# Autodesk Inventor assembly: CMV12000 Extraction Tool V01
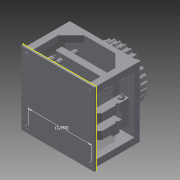
[picture p0: Inventor's stored thumbnail of the model, 180x180]
Saved by Autodesk Inventor 2015 (Build 190159000, 159)
## iProperties
Created: 2016-09-16
Part Number: CMV12000 Extraction Tool V01
Document SubType Name: Assembly
Designer: spichelh
Author: spichelh
## Documents named in this file (7)
- C:\Users\spichelh\Documents\GitHub\beta-hardware\Manufacturing Tools\CMV12000 Extraction Tool V01\CMV12000 Extraction Tool V01.iam
- C:\Users\spichelh\Documents\GitHub\beta-hardware\Manufacturing Tools\CMV12000 Extraction Tool V01\CMV12000v1.ipt
- C:\Users\spichelh\Documents\GitHub\beta-hardware\Manufacturing Tools\CMV12000 Extraction Tool V01\arms01.ipt
- C:\Users\spichelh\Documents\GitHub\beta-hardware\Manufacturing Tools\CMV12000 Extraction Tool V01\base.ipt
- C:\Users\spichelh\Documents\GitHub\beta-hardware\Manufacturing Tools\CMV12000 Extraction Tool V01\mover01.ipt
- C:\Users\spichelh\Documents\GitHub\beta-hardware\Manufacturing Tools\CMV12000 Extraction Tool V01\Knob01.ipt
- C:\Users\spichelh\Documents\GitHub\beta-hardware\Manufacturing Tools\CMV12000 Extraction Tool V01\SFE PCB.ipt
## Components (9 placed, 6 different names)
1. CMV12000v1:1 — Flush:8, Flush:9, Mate:7, Mate:11, Mate:14, Mate:15, Mate:16, Mate:17
2. arms01:1 — Rotational:2, Mate:14
3. arms01:2 — Mate:11, Rotational:5
4. base:1 — Flush:8, Flush:9, Mate:7, Mate:8, Mate:9, Mate:10, Mate:12, Mate:20, Mate:21, Mate:22
5. arms01:3 — Mate:16, Rotational:3
6. arms01:4 — Rotational:4, Mate:17
7. mover01:1 — Mate:8, Mate:9, Mate:10, Mate:13, Rotational:2, Rotational:3, Rotational:4, Rotational:5
8. Knob01:1 — Mate:12, Mate:13
9. SFE PCB:1 — Mate:15, Mate:18, Mate:19, Flush:10, Mate:20, Mate:21, Mate:22
## Relationships (23: Mate 16, RevoluteJoint 4, Flush 3)
- Flush:8 (-3 mm): CMV12000v1:1 ↔ base:1
- Flush:9 (-1 mm): CMV12000v1:1 ↔ base:1
- Mate:7 (1 mm): CMV12000v1:1 ↔ base:1
- Mate:8: base:1 ↔ mover01:1
- Mate:9: base:1 ↔ mover01:1
- Mate:10 (7 mm): base:1 ↔ mover01:1
- Mate:11: CMV12000v1:1 ↔ arms01:2
- Mate:12: base:1 ↔ Knob01:1
- Mate:13: mover01:1 ↔ Knob01:1
- Rotational:2 [RevoluteJoint]: arms01:1 ↔ mover01:1
- Mate:14: CMV12000v1:1 ↔ arms01:1
- Mate:15 (4 mm): CMV12000v1:1 ↔ SFE PCB:1
- Mate:16: CMV12000v1:1 ↔ arms01:3
- Rotational:3 [RevoluteJoint]: arms01:3 ↔ mover01:1
- Rotational:4 [RevoluteJoint]: arms01:4 ↔ mover01:1
- Mate:17: CMV12000v1:1 ↔ arms01:4
- Rotational:5 [RevoluteJoint]: arms01:2 ↔ mover01:1
- Mate:18: SFE PCB:1
- Mate:19: SFE PCB:1
- Flush:10: SFE PCB:1
- Mate:20: base:1 ↔ SFE PCB:1
- Mate:21: base:1 ↔ SFE PCB:1
- Mate:22: base:1 ↔ SFE PCB:1
